# Autodesk Inventor assembly: 12mm_Tube_Connector
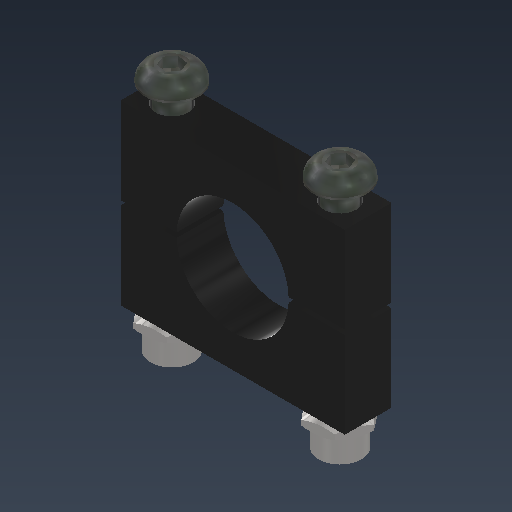
[picture p0: Inventor's stored thumbnail of the model, 512x512]
Saved by Autodesk Inventor 2024.1 (Build 281209000, 209)
## iProperties
Created: 2023-12-07
Part Number: 12mm_Tube_Connector
Document SubType Name: Assembly
Designer: dzw04
Mass: 5.539 g
Surface Area: 26.0043 cm^2
Volume: 1.85473 cm^3
Density: 2.98641 g/cm^3
Author: dzw04
## Documents named in this file (5)
- C:\Users\dzw04\OneDrive - Saxion\General - Mechatronica Lectoraat LMECH LED\Database ARG\Component_Database\SARAX\01. CAD\01. 3D_Drawing\02. Sub_Assemblies\Battery_Tray\02. Sub_Assemblies\12mm_Tube_Connector.iam
- C:\Users\dzw04\OneDrive - Saxion\General - Mechatronica Lectoraat LMECH LED\Database ARG\Component_Database\SARAX\01. CAD\01. 3D_Drawing\02. Sub_Assemblies\Battery_Tray\01. Parts\12mm_Tube_Connecotor.ipt
- C:\Users\dzw04\OneDrive - Saxion\General - Mechatronica Lectoraat LMECH LED\Database ARG\Component_Database\SARAX\01. CAD\01. 3D_Drawing\01. Parts\en-US\ISO 7380-1\ISO 7380-1 - M3 x 25.ipt
- C:\Users\dzw04\OneDrive - Saxion\General - Mechatronica Lectoraat LMECH LED\Database ARG\Component_Database\SARAX\01. CAD\01. 3D_Drawing\01. Parts\en-US\ISO 10511\ISO 10511 - M3.ipt
- C:\Users\dzw04\OneDrive - Saxion\General - Mechatronica Lectoraat LMECH LED\Database ARG\Component_Database\SARAX\01. CAD\01. 3D_Drawing\Parameters.xlsx
## Components (6 placed, 3 different names)
1. 12mm_Tube_Connecotor:1 — Flush:1, Flush:2, Mate:1, Mate:2, Mate:3
2. 12mm_Tube_Connecotor:2 — Flush:1, Flush:2, Mate:1, Mate:5
3. ISO 7380-1 M3 x 25:1 — Mate:4, Mate:5
4. DIN EN ISO 10511 M3:1 — Mate:2, Mate:3, Mate:4
5. ISO 7380-1 M3 x 25:2
6. DIN EN ISO 10511 M3:2
## Component patterns: (2 elements, first: ISO 7380-1 M3 x 25:1 + DIN EN ISO 10511 M3:1)
## Relationships (7: Mate 5, Flush 2)
- Flush:1: 12mm_Tube_Connecotor:1 ↔ 12mm_Tube_Connecotor:2
- Flush:2: 12mm_Tube_Connecotor:1 ↔ 12mm_Tube_Connecotor:2
- Mate:1 (0.5 mm): 12mm_Tube_Connecotor:1 ↔ 12mm_Tube_Connecotor:2
- Mate:2: 12mm_Tube_Connecotor:1 ↔ DIN EN ISO 10511 M3:1
- Mate:3: 12mm_Tube_Connecotor:1 ↔ DIN EN ISO 10511 M3:1
- Mate:4: ISO 7380-1 M3 x 25:1 ↔ DIN EN ISO 10511 M3:1
- Mate:5 (2 mm): 12mm_Tube_Connecotor:2 ↔ ISO 7380-1 M3 x 25:1
## Named parameters: NumberOfArms = 4, RotorToRotor = 900 mm, MountToMotorCenter = 0 mm, ArmPosition = 5 deg, LoadpipeLength = 450 mm, NumberOfBatterys = 2, BatteryLength = 200 mm, BatteryWidth = 62 mm, BatteryHeight = 76 mm, ThicknessBodyOuterPlate = 2 mm, ThicknessBodyCenterPlate = 2 mm, ThicknessLegLoadpipePlate = 2 mm, ThicknessBatteryTray = 2 mm, ThicknessBatteryTopTray = 1 mm, LandingGearHeight = 400 mm, LandingGearStabilityBar = 525 mm, LandingGearRod = 390 mm, StartAngleArm = 45 deg, MotorMountCenter = 71.5 mm
